# Autodesk Inventor assembly: Ensamblaje
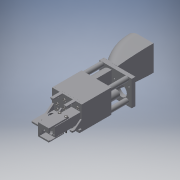
[picture p0: Inventor's stored thumbnail of the model, 180x180]
Saved by Autodesk Inventor 2019 (Build 230136000, 136)
## iProperties
Created: 2020-09-07
Part Number: Ensamblaje
Document SubType Name: Assembly
Designer: ASUS
Author: ASUS
## Documents named in this file (11)
- C:\Users\ASUS\Documents\Life\College\Graduation Project\Ensamblaje.iam
- C:\Users\ASUS\Documents\Life\College\Graduation Project\Plate.ipt
- C:\Users\ASUS\Documents\Life\College\Graduation Project\Bowl.ipt
- C:\Users\ASUS\Documents\Life\College\Graduation Project\Motor.ipt
- C:\Users\ASUS\Documents\Life\College\Graduation Project\Screw.ipt
- C:\Users\ASUS\Documents\Life\College\Graduation Project\heatblock.ipt
- C:\Users\ASUS\Documents\Life\College\Graduation Project\FeedExtension.ipt
- C:\Users\ASUS\Documents\Life\College\Graduation Project\HeatHolder.ipt
- C:\Users\ASUS\Documents\Inventor\Content Center Files\R2019\en-US\BS EN ISO 7045 Z\EN ISO 7045 - M3 x 20 - 4.8 - Z(1).ipt
- C:\Users\ASUS\Documents\Inventor\Content Center Files\R2019\en-US\AS 1427(05)\AS 1427 - M3 x 30(5) II.ipt
- C:\Users\ASUS\Documents\Inventor\Content Center Files\R2019\en-US\AS 1427(05)\AS 1427 - M3 x 8(5) II.ipt
## Components (22 placed, 10 different names)
1. Plate:1 — Flush:3, Flush:4, Mate:7, Mate:11, Insert:1, Insert:2, Mate:25, Mate:26, Mate:27, Mate:28, Mate:29, Mate:30, Mate:31, Mate:32, Mate:33, Mate:34, Mate:35, Mate:36, Mate:37, Mate:38, Mate:39, Mate:40
2. Bowl:1 — Flush:3, Flush:4, Flush:5, Flush:6, Mate:5, Mate:7, Mate:10
3. Motor:1 — Flush:5, Flush:6, Mate:4, Mate:5, Mate:6, Mate:9, Flush:7, Flush:8, Mate:19, Mate:20
4. Screw:1 — Mate:4, Mate:6, Mate:8
5. heatblock:1 — Mate:8, Mate:10, Mate:11, Mate:12, Mate:13, Mate:14, Mate:21
6. FeedExtension:1 — Mate:9, Flush:7, Flush:8, Mate:15, Mate:16, Mate:17, Mate:18
7. HeatHolder:1 — Mate:12, Mate:13, Mate:14, Mate:22, Mate:23, Mate:24
8. BS EN ISO 7045 Z - Metric M3 x 20 - 4.8 - Z:1 — Mate:15, Mate:16
9. BS EN ISO 7045 Z - Metric M3 x 20 - 4.8 - Z:2 — Mate:17, Mate:18
10. BS EN ISO 7045 Z - Metric M3 x 20 - 4.8 - Z:3 — Mate:19, Mate:20
11. AS 1427 H - Metric M3 x 30:1 — Mate:21, Mate:22
12. AS 1427 H - Metric M3 x 30:2 — Mate:23, Mate:24
13. AS 1427 H - Metric M3 x 8:2 — Insert:1
14. AS 1427 H - Metric M3 x 8:1 — Insert:2
15. AS 1427 H - Metric M3 x 8:3 — Mate:25, Mate:26
16. AS 1427 H - Metric M3 x 8:5 — Mate:27, Mate:28
17. AS 1427 H - Metric M3 x 8:7 — Mate:29, Mate:30
18. AS 1427 H - Metric M3 x 8:10 — Mate:31, Mate:32
19. AS 1427 H - Metric M3 x 8:9 — Mate:33, Mate:34
20. AS 1427 H - Metric M3 x 8:6 — Mate:35, Mate:36
21. AS 1427 H - Metric M3 x 8:4 — Mate:37, Mate:38
22. AS 1427 H - Metric M3 x 8:8 — Mate:39, Mate:40
## Relationships (45: Mate 37, Flush 6, Insert 2)
- Flush:3: Plate:1 ↔ Bowl:1
- Flush:4: Plate:1 ↔ Bowl:1
- Flush:5: Bowl:1 ↔ Motor:1
- Flush:6: Bowl:1 ↔ Motor:1
- Mate:4: Motor:1 ↔ Screw:1
- Mate:5: Bowl:1 ↔ Motor:1
- Mate:6 (10.5 mm): Motor:1 ↔ Screw:1
- Mate:7: Plate:1 ↔ Bowl:1
- Mate:8: Screw:1 ↔ heatblock:1
- Mate:9: Motor:1 ↔ FeedExtension:1
- Flush:7: Motor:1 ↔ FeedExtension:1
- Flush:8: Motor:1 ↔ FeedExtension:1
- Mate:10: Bowl:1 ↔ heatblock:1
- Mate:11 (3 mm): Plate:1 ↔ heatblock:1
- Mate:12: heatblock:1 ↔ HeatHolder:1
- Mate:13: heatblock:1 ↔ HeatHolder:1
- Mate:14 (1 mm): heatblock:1 ↔ HeatHolder:1
- Mate:15: FeedExtension:1 ↔ BS EN ISO 7045 Z - Metric M3 x 20 - 4.8 - Z:1
- Mate:16: FeedExtension:1 ↔ BS EN ISO 7045 Z - Metric M3 x 20 - 4.8 - Z:1
- Mate:17: FeedExtension:1 ↔ BS EN ISO 7045 Z - Metric M3 x 20 - 4.8 - Z:2
- Mate:18: FeedExtension:1 ↔ BS EN ISO 7045 Z - Metric M3 x 20 - 4.8 - Z:2
- Mate:19: Motor:1 ↔ BS EN ISO 7045 Z - Metric M3 x 20 - 4.8 - Z:3
- Mate:20: Motor:1 ↔ BS EN ISO 7045 Z - Metric M3 x 20 - 4.8 - Z:3
- Mate:21: heatblock:1 ↔ AS 1427 H - Metric M3 x 30:1
- Mate:22: HeatHolder:1 ↔ AS 1427 H - Metric M3 x 30:1
- Mate:23: HeatHolder:1 ↔ AS 1427 H - Metric M3 x 30:2
- Mate:24: HeatHolder:1 ↔ AS 1427 H - Metric M3 x 30:2
- Insert:1: Plate:1 ↔ AS 1427 H - Metric M3 x 8:2
- Insert:2: Plate:1 ↔ AS 1427 H - Metric M3 x 8:1
- Mate:25: Plate:1 ↔ AS 1427 H - Metric M3 x 8:3
- Mate:26: Plate:1 ↔ AS 1427 H - Metric M3 x 8:3
- Mate:27: Plate:1 ↔ AS 1427 H - Metric M3 x 8:5
- Mate:28: Plate:1 ↔ AS 1427 H - Metric M3 x 8:5
- Mate:29: Plate:1 ↔ AS 1427 H - Metric M3 x 8:7
- Mate:30: Plate:1 ↔ AS 1427 H - Metric M3 x 8:7
- Mate:31: Plate:1 ↔ AS 1427 H - Metric M3 x 8:10
- Mate:32: Plate:1 ↔ AS 1427 H - Metric M3 x 8:10
- Mate:33: Plate:1 ↔ AS 1427 H - Metric M3 x 8:9
- Mate:34: Plate:1 ↔ AS 1427 H - Metric M3 x 8:9
- Mate:35: Plate:1 ↔ AS 1427 H - Metric M3 x 8:6
- Mate:36: Plate:1 ↔ AS 1427 H - Metric M3 x 8:6
- Mate:37: Plate:1 ↔ AS 1427 H - Metric M3 x 8:4
- Mate:38: Plate:1 ↔ AS 1427 H - Metric M3 x 8:4
- Mate:39: Plate:1 ↔ AS 1427 H - Metric M3 x 8:8
- Mate:40: Plate:1 ↔ AS 1427 H - Metric M3 x 8:8
